# Autodesk Inventor assembly: FloatingIntake2
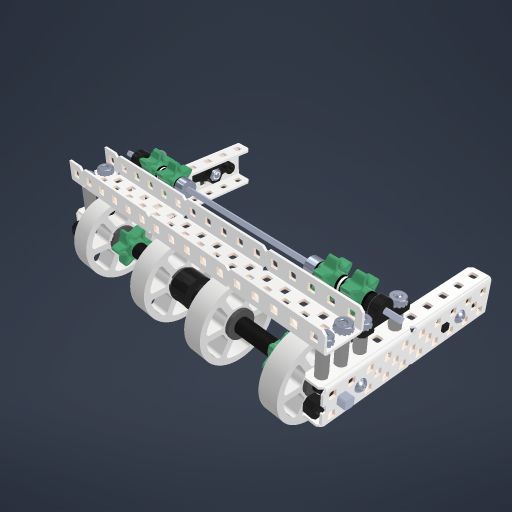
[picture p0: Inventor's stored thumbnail of the model, 512x512]
Saved by Autodesk Inventor 2023 (Build 270158000, 158)
## iProperties
Created: 2022-10-30
Part Number: FloatingIntake2
Document SubType Name: Assembly
Designer: alex
Author: alex
## Documents named in this file (33)
- C:\Users\alex\Documents\GitHub\4067X_spin_up_cad\FloatingIntake2.iam
- C:\Users\alex\Documents\GitHub\4067X_spin_up_cad\WithAdapter2Inch.iam
- C:\Users\alex\Documents\GitHub\4067X_spin_up_cad\Library\Structure\C-Channels\Aluminum 1x2x1\Alu C 1x2x1x10.ipt
- C:\Users\alex\Documents\GitHub\4067X_spin_up_cad\Library\Structure\Standoff.ipt
- C:\Users\alex\Documents\GitHub\4067X_spin_up_cad\Library\Structure\C-Channels\Aluminum 1x2x1\Alu C 1x2x1x16.ipt
- C:\Users\alex\Documents\GitHub\4067X_spin_up_cad\Library\Motion\Sprockets\HS 6T Sprocket, No Insert.ipt
- C:\Users\alex\Documents\GitHub\4067X_spin_up_cad\Library\Motion\Shaft HS\Shaft HS\Shaft HS 8.5 in.ipt
- C:\Users\alex\Documents\GitHub\4067X_spin_up_cad\Library\Motion\Shaft HS\Shaft HS.ipt
- C:\Users\alex\Documents\GitHub\4067X_spin_up_cad\Library\Motion\Shaft HS\HS Bearing Flat.ipt
- C:\Users\alex\Documents\GitHub\4067X_spin_up_cad\Library\Structure\Hardware\Screw Steel - Star\SScrew Star Smooth .500.ipt
- C:\Users\alex\Documents\GitHub\4067X_spin_up_cad\Library\Structure\Hardware\Screw Steel - Star.ipt
- C:\Users\alex\Documents\GitHub\4067X_spin_up_cad\Library\Structure\Hardware\Nut Thin Nylock.ipt
- C:\Users\alex\Documents\GitHub\4067X_spin_up_cad\Library\Motion\1-Post Bearing Flat Hex Retainer.ipt
- C:\Users\alex\Documents\GitHub\4067X_spin_up_cad\Library\Structure\Hardware\Nut Nylock.ipt
- C:\Users\alex\Documents\GitHub\4067X_spin_up_cad\Library\Structure\Hardware\Screw Steel - Star\SScrew Star Smooth .375.ipt
- C:\Users\alex\Documents\GitHub\4067X_spin_up_cad\Library\Motion\Shaft HS\HS Spacer\HSpacer .1250.ipt
- C:\Users\alex\Documents\GitHub\4067X_spin_up_cad\Library\Motion\Shaft HS\HS Spacer.ipt
- C:\Users\alex\Documents\GitHub\4067X_spin_up_cad\Library\Structure\Hardware\Nut Keps.ipt
- C:\Users\alex\Documents\GitHub\4067X_spin_up_cad\Library\Structure\Standoff\Standoff .50.ipt
- C:\Users\alex\Documents\GitHub\4067X_spin_up_cad\Library\Motion\Pillow Bearing Block.ipt
- C:\Users\alex\Documents\GitHub\4067X_spin_up_cad\Library\Motion\Shaft LS\Shaft LS 8.5 in.ipt
- C:\Users\alex\Documents\GitHub\4067X_spin_up_cad\Library\Motion\Shaft LS.ipt
- C:\Users\alex\Documents\GitHub\4067X_spin_up_cad\Library\Motion\Sprockets\HS 6T Sprocket, Square.ipt
- C:\Users\alex\Documents\GitHub\4067X_spin_up_cad\Library\Motion\Spacers\Spacer Nylon .375 OD\NSpacer .375 OD x .125.ipt
- C:\Users\alex\Documents\GitHub\4067X_spin_up_cad\Library\Motion\Spacers\Spacer Nylon .375 OD.ipt
- C:\Users\alex\Documents\GitHub\4067X_spin_up_cad\Library\Motion\Spacers\Washer Teflon\TWasher .375 OD x .06250.ipt
- C:\Users\alex\Documents\GitHub\4067X_spin_up_cad\Library\Motion\Spacers\Washer Teflon.ipt
- C:\Users\alex\Documents\GitHub\4067X_spin_up_cad\Library\Motion\Shaft Collar with Set Screw.ipt
- C:\Users\alex\Documents\GitHub\4067X_spin_up_cad\Library\Motion\Shaft HS\HS Spacer\HSpacer .5000.ipt
- C:\Users\alex\Documents\GitHub\4067X_spin_up_cad\Library\Motion\Shaft HS\HS Shaft Collar.ipt
- C:\Users\alex\Documents\GitHub\4067X_spin_up_cad\Library\Structure\Standoff\Standoff .75.ipt
- C:\Users\alex\Documents\GitHub\4067X_spin_up_cad\Library\Structure\Hardware\Screw Steel - Star\SScrew Star Smooth 1.000.ipt
- C:\Users\alex\Documents\GitHub\4067X_spin_up_cad\Library\Structure\Hardware\Screw Steel - Star\SScrew Star Smooth .875.ipt
## Components (67 placed, 25 different names)
1. WithAdapter2Inch:1 [sub-assembly] — Insert:34, Insert:35
2. Alu C 1x2x1x10:1 — Flush:1, Insert:38, Insert:39, Flush:4, Insert:77, Insert:78, Insert:83, Insert:84, Insert:90, Insert:91
3. Alu C 1x2x1x10:2 — Flush:1, Insert:21, Mate:6, Insert:22, Insert:42, Insert:43, Flush:4, Insert:73, Insert:74, Insert:75, Insert:76, Insert:85, Insert:86
4. Shaft HS 8.5 in:1
5. HS Bearing Flat:1 — Insert:17
6. SScrew Star Smooth .500:1
7. Nut Thin Nylock:1
8. 1-Post Bearing Flat Hex Retainer:1
9. Nut Nylock:1
10. SScrew Star Smooth .375:2
11. SScrew Star Smooth .375:3
12. Nut Nylock:2
13. 1-Post Bearing Flat Hex Retainer:2
14. HSpacer .1250:1 — Insert:17, Insert:34
15. HS Bearing Flat:2 — Insert:21, Mate:6, Insert:31
16. Nut Thin Nylock:2
17. SScrew Star Smooth .500:4 — Insert:22
18. Nut Keps:3 — Insert:82
19. Nut Keps:4 — Insert:81
20. HSpacer .1250:2 — Insert:31, Insert:36
21. WithAdapter2Inch:2 [sub-assembly] — Insert:36, Insert:37
22. HS 6T Sprocket, No Insert:3 — Insert:35, Insert:71
23. HS 6T Sprocket, No Insert:4 — Insert:37, Insert:66
24. Standoff .50:5 — Insert:38, Insert:40
25. Standoff .50:6 — Insert:39, Mate:7
26. Pillow Bearing Block:1 — Insert:40, Mate:7, Insert:58, Flush:3, Insert:81, Insert:82
27. Standoff .50:7 — Insert:42
28. Standoff .50:8 — Insert:43
29. Pillow Bearing Block:2 — Insert:61, Insert:87, Insert:88
30. Shaft LS 8.5 in:1 — Mate:9, Mate:10, Flush:3
31. TWasher .375 OD x .06250:1 — Insert:60, Insert:64
32. HS 6T Sprocket, Square:3 — Insert:53, Insert:57
33. Shaft Collar with Set Screw:2 — Insert:53
34. TWasher .375 OD x .06250:3 — Insert:57, Insert:63
35. NSpacer .375 OD x .125:3 — Insert:58, Insert:59
36. HS 6T Sprocket, Square:5 — Insert:59, Insert:60
37. NSpacer .375 OD x .125:4 — Insert:61, Insert:62
38. HS 6T Sprocket, Square:6 — Insert:62, Insert:63
39. HS 6T Sprocket, Square:7 — Mate:9, Mate:10, Insert:64, Insert:65
40. Shaft Collar with Set Screw:3 — Insert:65
41. HSpacer .5000:3 — Insert:66, Insert:67
42. HSpacer .5000:4 — Insert:67, Insert:68
43. WithAdapter2Inch:3 [sub-assembly] — Insert:68
44. HSpacer .5000:5 — Insert:71
45. HSpacer .5000:6
46. WithAdapter2Inch:4 [sub-assembly]
47. HS Shaft Collar:1
48. HS Shaft Collar:2
49. Alu C 1x2x1x16:1 — Insert:79, Insert:80, Insert:89, Insert:92, Insert:93, Insert:94
50. Standoff .75:9 — Insert:73, Insert:79
51. Standoff .75:10 — Insert:74
52. SScrew Star Smooth 1.000:8 — Insert:75
53. SScrew Star Smooth 1.000:9 — Insert:76
54. Standoff .75:11 — Insert:77
55. Standoff .75:12 — Insert:78, Insert:94
56. Nut Keps:5 — Insert:80
57. SScrew Star Smooth .875:10 — Insert:83
58. SScrew Star Smooth .875:11 — Insert:84
59. SScrew Star Smooth .875:12 — Insert:85
60. SScrew Star Smooth .875:13 — Insert:86
61. Nut Keps:6 — Insert:87
62. Nut Keps:7 — Insert:88
63. Nut Keps:8 — Insert:89
64. SScrew Star Smooth 1.000:14 — Insert:90
65. SScrew Star Smooth 1.000:15 — Insert:91
66. Nut Keps:9 — Insert:92
67. Nut Keps:10 — Insert:93
## Relationships (80: Insert 63, Mate 12, Flush 4, Angle 1)
- [Mate]: WithAdapter2Inch:1 ↔ Alu C 1x2x1x10:1
- [Angle] (0 deg): Alu C 1x2x1x10:1 ↔ Alu C 1x2x1x10:2
- Flush:1: Alu C 1x2x1x10:1 ↔ Alu C 1x2x1x10:2
- [Mate]: Alu C 1x2x1x10:2 ↔ Shaft HS 8.5 in:1
- [Flush] (-5.08 mm): Alu C 1x2x1x10:1 ↔ Shaft HS 8.5 in:1
- [Insert]: Alu C 1x2x1x10:1 ↔ HS Bearing Flat:1
- [Mate]: Alu C 1x2x1x10:1 ↔ HS Bearing Flat:1
- [Insert]: Alu C 1x2x1x10:1 ↔ SScrew Star Smooth .500:1
- [Insert]: HS Bearing Flat:1 ↔ Nut Thin Nylock:1
- [Insert]: 1-Post Bearing Flat Hex Retainer:1 ↔ Nut Nylock:1
- [Insert]: Alu C 1x2x1x10:2 ↔ 1-Post Bearing Flat Hex Retainer:1
- [Mate]: Alu C 1x2x1x10:2 ↔ 1-Post Bearing Flat Hex Retainer:1
- [Insert]: Alu C 1x2x1x10:2 ↔ SScrew Star Smooth .375:2
- [Insert]: Alu C 1x2x1x10:1 ↔ 1-Post Bearing Flat Hex Retainer:2
- [Mate]: Alu C 1x2x1x10:1 ↔ 1-Post Bearing Flat Hex Retainer:2
- [Insert]: Alu C 1x2x1x10:1 ↔ SScrew Star Smooth .375:3
- [Insert]: Nut Nylock:2 ↔ 1-Post Bearing Flat Hex Retainer:2
- Insert:17: HS Bearing Flat:1 ↔ HSpacer .1250:1
- [Insert]: HS Bearing Flat:2 ↔ Nut Thin Nylock:2
- Insert:21: Alu C 1x2x1x10:2 ↔ HS Bearing Flat:2
- Mate:6: Alu C 1x2x1x10:2 ↔ HS Bearing Flat:2
- Insert:22: Alu C 1x2x1x10:2 ↔ SScrew Star Smooth .500:4
- Insert:31: HS Bearing Flat:2 ↔ HSpacer .1250:2
- Insert:34: WithAdapter2Inch:1 ↔ HSpacer .1250:1
- Insert:35: WithAdapter2Inch:1 ↔ HS 6T Sprocket, No Insert:3
- Insert:36: HSpacer .1250:2 ↔ WithAdapter2Inch:2
- Insert:37: WithAdapter2Inch:2 ↔ HS 6T Sprocket, No Insert:4
- Insert:38: Alu C 1x2x1x10:1 ↔ Standoff .50:5
- Insert:39: Alu C 1x2x1x10:1 ↔ Standoff .50:6
- Insert:40: Standoff .50:5 ↔ Pillow Bearing Block:1
- Mate:7: Standoff .50:6 ↔ Pillow Bearing Block:1
- [Insert]: Standoff .50:7 ↔ Pillow Bearing Block:2
- [Mate]: Standoff .50:8 ↔ Pillow Bearing Block:2
- Insert:42: Alu C 1x2x1x10:2 ↔ Standoff .50:7
- Insert:43: Alu C 1x2x1x10:2 ↔ Standoff .50:8
- Insert:53: HS 6T Sprocket, Square:3 ↔ Shaft Collar with Set Screw:2
- Insert:57: HS 6T Sprocket, Square:3 ↔ TWasher .375 OD x .06250:3
- Insert:58: Pillow Bearing Block:1 ↔ NSpacer .375 OD x .125:3
- Insert:59: NSpacer .375 OD x .125:3 ↔ HS 6T Sprocket, Square:5
- Insert:60: TWasher .375 OD x .06250:1 ↔ HS 6T Sprocket, Square:5
- Insert:61: Pillow Bearing Block:2 ↔ NSpacer .375 OD x .125:4
- Insert:62: NSpacer .375 OD x .125:4 ↔ HS 6T Sprocket, Square:6
- Insert:63: TWasher .375 OD x .06250:3 ↔ HS 6T Sprocket, Square:6
- Mate:9: Shaft LS 8.5 in:1 ↔ HS 6T Sprocket, Square:7
- Mate:10: Shaft LS 8.5 in:1 ↔ HS 6T Sprocket, Square:7
- Insert:64: TWasher .375 OD x .06250:1 ↔ HS 6T Sprocket, Square:7
- Flush:3 (-9.525 mm): Pillow Bearing Block:1 ↔ Shaft LS 8.5 in:1
- Insert:65: HS 6T Sprocket, Square:7 ↔ Shaft Collar with Set Screw:3
- Insert:66: HS 6T Sprocket, No Insert:4 ↔ HSpacer .5000:3
- Insert:67: HSpacer .5000:3 ↔ HSpacer .5000:4
- Insert:68: HSpacer .5000:4 ↔ WithAdapter2Inch:3
- [Insert]: HSpacer .5000:5 ↔ HSpacer .5000:6
- [Insert]: HSpacer .5000:6 ↔ WithAdapter2Inch:4
- Insert:71: HS 6T Sprocket, No Insert:3 ↔ HSpacer .5000:5
- [Mate]: Shaft HS 8.5 in:1 ↔ HS Shaft Collar:1
- [Mate]: WithAdapter2Inch:4 ↔ HS Shaft Collar:1
- [Insert]: WithAdapter2Inch:3 ↔ HS Shaft Collar:2
- Flush:4: Alu C 1x2x1x10:1 ↔ Alu C 1x2x1x10:2
- Insert:73: Alu C 1x2x1x10:2 ↔ Standoff .75:9
- Insert:74: Alu C 1x2x1x10:2 ↔ Standoff .75:10
- Insert:75: Alu C 1x2x1x10:2 ↔ SScrew Star Smooth 1.000:8
- Insert:76: Alu C 1x2x1x10:2 ↔ SScrew Star Smooth 1.000:9
- Insert:77: Alu C 1x2x1x10:1 ↔ Standoff .75:11
- Insert:78: Alu C 1x2x1x10:1 ↔ Standoff .75:12
- Insert:79: Alu C 1x2x1x16:1 ↔ Standoff .75:9
- Insert:80: Alu C 1x2x1x16:1 ↔ Nut Keps:5
- Insert:81: Nut Keps:4 ↔ Pillow Bearing Block:1
- Insert:82: Nut Keps:3 ↔ Pillow Bearing Block:1
- Insert:83: Alu C 1x2x1x10:1 ↔ SScrew Star Smooth .875:10
- Insert:84: Alu C 1x2x1x10:1 ↔ SScrew Star Smooth .875:11
- Insert:85: Alu C 1x2x1x10:2 ↔ SScrew Star Smooth .875:12
- Insert:86: Alu C 1x2x1x10:2 ↔ SScrew Star Smooth .875:13
- Insert:87: Pillow Bearing Block:2 ↔ Nut Keps:6
- Insert:88: Pillow Bearing Block:2 ↔ Nut Keps:7
- Insert:89: Alu C 1x2x1x16:1 ↔ Nut Keps:8
- Insert:90: Alu C 1x2x1x10:1 ↔ SScrew Star Smooth 1.000:14
- Insert:91: Alu C 1x2x1x10:1 ↔ SScrew Star Smooth 1.000:15
- Insert:92: Alu C 1x2x1x16:1 ↔ Nut Keps:9
- Insert:93: Alu C 1x2x1x16:1 ↔ Nut Keps:10
- Insert:94: Alu C 1x2x1x16:1 ↔ Standoff .75:12
## Named parameters: d174_d168 = 0 mm, d27_d182 = 0 mm, d51_d49 = 0 mm, d52_d50 = 0 mm, d85_d83 = 0 mm, d86_d84 = 0 mm
